# Autodesk Inventor assembly: R2_D2
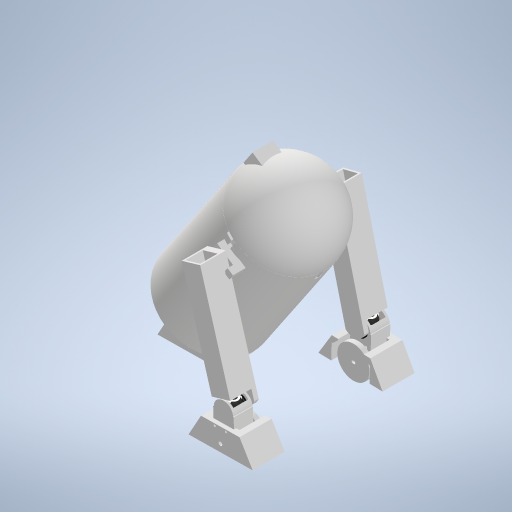
[picture p0: Inventor's stored thumbnail of the model, 512x512]
Saved by Autodesk Inventor 2024 (Build 280153000, 153)
## iProperties
Created: 2025-06-20
Part Number: R2_D2
Document SubType Name: Assembly
Designer: Aidan
Author: Aidan
## Documents named in this file (14)
- C:\Users\Aidan\OneDrive - University of New Haven\Documents\Fun Coding\R2-D2_V1\3D_Models\R2_D2.iam
- C:\Users\Aidan\OneDrive - University of New Haven\Documents\Fun Coding\R2-D2_V1\3D_Models\Wheel_well.ipt
- C:\Users\Aidan\OneDrive - University of New Haven\Documents\Fun Coding\R2-D2_V1\3D_Models\Skate-Bearing\Skate-Bearing.ipt
- C:\Users\Aidan\OneDrive - University of New Haven\Documents\Fun Coding\R2-D2_V1\3D_Models\Mini Gear DC Motor 6 V Yellow\Mini Gear DC Motor 6 V Yellow.ipt
- C:\Users\Aidan\OneDrive - University of New Haven\Documents\Fun Coding\R2-D2_V1\3D_Models\Wheel.ipt
- C:\Users\Aidan\OneDrive - University of New Haven\Documents\Fun Coding\R2-D2_V1\3D_Models\motor_mount.ipt
- C:\Users\Aidan\OneDrive - University of New Haven\Documents\Fun Coding\R2-D2_V1\3D_Models\arm1.ipt
- C:\Users\Aidan\OneDrive - University of New Haven\Documents\Fun Coding\R2-D2_V1\3D_Models\main_body.ipt
- C:\Users\Aidan\OneDrive - University of New Haven\Documents\Fun Coding\R2-D2_V1\3D_Models\center_wheel_well.ipt
- C:\Users\Aidan\OneDrive - University of New Haven\Documents\Fun Coding\R2-D2_V1\3D_Models\middle_wheel.ipt
- C:\Users\Aidan\OneDrive - University of New Haven\Documents\Fun Coding\R2-D2_V1\3D_Models\middle_pivot_axel.ipt
- C:\Users\Aidan\OneDrive - University of New Haven\Documents\Fun Coding\R2-D2_V1\3D_Models\middle_wheel_axel.ipt
- C:\Users\Aidan\OneDrive - University of New Haven\Documents\Fun Coding\R2-D2_V1\3D_Models\dome.ipt
- C:\Users\Aidan\OneDrive - University of New Haven\Documents\Fun Coding\R2-D2_V1\3D_Models\c270_webcam\logitech_webcam_c270\logitech_webcam_c270.ipt
## Components (23 placed, 13 different names)
1. Wheel_well:1 — Flush:5, Mate:4, Mate:6, Mate:7
2. Mini Gear DC Motor 6 V Yellow:1 — Mate:2, Flush:5, Mate:5, Mate:6, Mate:7, Mate:9
3. Wheel:1 — Mate:2
4. Skate-Bearing:1 — Rotational:1, Insert:9
5. motor_mount:1 — Mate:4, Mate:5, Mate:9, Insert:9
6. arm1:1 — Rotational:1, Rotational:2
7. main_body:1 — Insert:2, Insert:3, Insert:13, Insert:17
8. Skate-Bearing:2 — Insert:2, Rotational:2
9. Skate-Bearing:3 — Insert:3, Rotational:3
10. Skate-Bearing:5 — Insert:13, Rotational:6
11. arm1:2 — Rotational:3, Rotational:4
12. Mini Gear DC Motor 6 V Yellow:2 — Insert:10, Insert:11, Mate:11, Mate:12
13. Wheel_well:2 — Insert:10, Mate:10
14. Wheel:2 — Insert:11
15. motor_mount:2 — Mate:10, Mate:11, Mate:12, Insert:12
16. Skate-Bearing:6 — Insert:12, Rotational:4
17. center_wheel_well:1 — Insert:15, Insert:16
18. middle_wheel:1 — Insert:14
19. Skate-Bearing:7 — Insert:14, Rotational:5
20. middle_pivot_axel:1 — Rotational:6, Insert:16
21. middle_wheel_axel:1 — Rotational:5, Insert:15
22. dome:1 — Insert:17, Insert:18
23. logitech_webcam_c270:1 — Insert:18
## Relationships (28: Insert 12, Mate 9, RevoluteJoint 6, Flush 1)
- Mate:2: Mini Gear DC Motor 6 V Yellow:1 ↔ Wheel:1
- Flush:5 (2.4 mm): Wheel_well:1 ↔ Mini Gear DC Motor 6 V Yellow:1
- Mate:4 (1 mm): Wheel_well:1 ↔ motor_mount:1
- Mate:5: Mini Gear DC Motor 6 V Yellow:1 ↔ motor_mount:1
- Mate:6: Wheel_well:1 ↔ Mini Gear DC Motor 6 V Yellow:1
- Rotational:1 [RevoluteJoint]: Skate-Bearing:1 ↔ arm1:1
- Mate:7 (2 mm): Wheel_well:1 ↔ Mini Gear DC Motor 6 V Yellow:1
- Insert:2: main_body:1 ↔ Skate-Bearing:2
- Rotational:2 [RevoluteJoint]: arm1:1 ↔ Skate-Bearing:2
- Insert:3: main_body:1 ↔ Skate-Bearing:3
- Rotational:3 [RevoluteJoint]: Skate-Bearing:3 ↔ arm1:2
- Mate:9 (1 mm): Mini Gear DC Motor 6 V Yellow:1 ↔ motor_mount:1
- Insert:9 (2 mm): Skate-Bearing:1 ↔ motor_mount:1
- Insert:10 (2 mm): Mini Gear DC Motor 6 V Yellow:2 ↔ Wheel_well:2
- Insert:11: Mini Gear DC Motor 6 V Yellow:2 ↔ Wheel:2
- Mate:10 (1 mm): Wheel_well:2 ↔ motor_mount:2
- Mate:11 (1 mm): Mini Gear DC Motor 6 V Yellow:2 ↔ motor_mount:2
- Mate:12 (0.85 mm): Mini Gear DC Motor 6 V Yellow:2 ↔ motor_mount:2
- Insert:12: motor_mount:2 ↔ Skate-Bearing:6
- Rotational:4 [RevoluteJoint]: arm1:2 ↔ Skate-Bearing:6
- Insert:13 (-2 mm): main_body:1 ↔ Skate-Bearing:5
- Insert:14 (-1 mm): middle_wheel:1 ↔ Skate-Bearing:7
- Rotational:5 [RevoluteJoint]: Skate-Bearing:7 ↔ middle_wheel_axel:1
- Insert:15: center_wheel_well:1 ↔ middle_wheel_axel:1
- Rotational:6 [RevoluteJoint]: Skate-Bearing:5 ↔ middle_pivot_axel:1
- Insert:16: center_wheel_well:1 ↔ middle_pivot_axel:1
- Insert:17: main_body:1 ↔ dome:1
- Insert:18 (25 mm): dome:1 ↔ logitech_webcam_c270:1
